# Autodesk Inventor assembly: Cycloidal Drive 1 - My Assembly
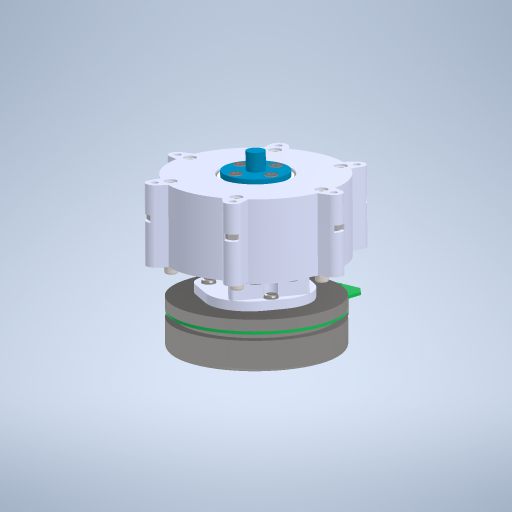
[picture p0: Inventor's stored thumbnail of the model, 512x512]
Saved by Autodesk Inventor 2023.2 (Build 272271000, 271)
## iProperties
Created: 2023-01-18
Part Number: Cycloidal Drive 1 - My Assembly
Document SubType Name: Assembly
Designer: Letícia
Author: Letícia
## Documents named in this file (31)
- C:\Users\User\Desktop\IC - Prof. Rafael\CADs\Redução Cicloidal\HowToMechatronics\Cycloidal Drive R25 - 3D\Cycloidal Drive - My Assembly.iam
- C:\Users\User\Desktop\IC - Prof. Rafael\CADs\Redução Cicloidal\HowToMechatronics\Cycloidal Drive R25 - 3D\Eccentric shaft v3.ipt
- C:\Users\User\Desktop\IC - Prof. Rafael\CADs\Redução Cicloidal\HowToMechatronics\Cycloidal Drive R25 - 3D\Ball Bearing-17x26x5mm.ipt
- C:\Users\User\Desktop\IC - Prof. Rafael\CADs\Redução Cicloidal\HowToMechatronics\Cycloidal Drive R25 - 3D\Ball Bearing-15x24x5mm 1.ipt
- C:\Users\User\Desktop\IC - Prof. Rafael\CADs\Redução Cicloidal\HowToMechatronics\Cycloidal Drive R25 - 3D\Distance ring 2.ipt
- C:\Users\User\Desktop\IC - Prof. Rafael\CADs\Redução Cicloidal\HowToMechatronics\Cycloidal Drive R25 - 3D\Cycloidal Disk v3 -.ipt
- C:\Users\User\Desktop\IC - Prof. Rafael\CADs\Redução Cicloidal\HowToMechatronics\Cycloidal Drive R25 - 3D\Output shaft p1 v3.ipt
- C:\Users\User\Desktop\IC - Prof. Rafael\CADs\Redução Cicloidal\HowToMechatronics\Cycloidal Drive R25 - 3D\Output shaft v3.ipt
- C:\Users\User\Desktop\IC - Prof. Rafael\CADs\Redução Cicloidal\HowToMechatronics\Cycloidal Drive R25 - 3D\Bushing 6x8mm.ipt
- C:\Users\User\Desktop\IC - Prof. Rafael\CADs\Redução Cicloidal\HowToMechatronics\Cycloidal Drive R25 - 3D\Pin 6x22mm r1.ipt
- C:\Users\User\Desktop\IC - Prof. Rafael\CADs\Redução Cicloidal\HowToMechatronics\Cycloidal Drive R25 - 3D\Input shaft 1 v3.ipt
- C:\Users\User\Desktop\IC - Prof. Rafael\CADs\Redução Cicloidal\HowToMechatronics\Cycloidal Drive R25 - 3D\Threaded insert M3 v3.ipt
- C:\Users\User\Desktop\IC - Prof. Rafael\CADs\Redução Cicloidal\HowToMechatronics\Cycloidal Drive R25 - 3D\porca prisioneiro.ipt
- C:\Users\User\Desktop\IC - Prof. Rafael\CADs\Redução Cicloidal\HowToMechatronics\Cycloidal Drive R25 - 3D\parafuso prisioneiro.ipt
- C:\Users\User\Desktop\IC - Prof. Rafael\CADs\Redução Cicloidal\HowToMechatronics\Cycloidal Drive R25 - 3D\EN ISO 4762 M3 x 25 - 18N_EN ISO 4762 M3 x 25 - 18N.ipt
- C:\Users\User\Desktop\IC - Prof. Rafael\CADs\Redução Cicloidal\HowToMechatronics\Cycloidal Drive R25 - 3D\Base housing.ipt
- C:\Users\User\Desktop\IC - Prof. Rafael\CADs\Redução Cicloidal\HowToMechatronics\Cycloidal Drive R25 - 3D\Pin 6x30mm r1.ipt
- C:\Users\User\Desktop\IC - Prof. Rafael\CADs\Redução Cicloidal\HowToMechatronics\Cycloidal Drive R25 - 3D\Ball Bearing-35x47x7mm 2.ipt
- C:\Users\User\Desktop\IC - Prof. Rafael\CADs\Redução Cicloidal\HowToMechatronics\Cycloidal Drive R25 - 3D\Housing lid.ipt
- C:\Users\User\Desktop\IC - Prof. Rafael\CADs\Redução Cicloidal\HowToMechatronics\Cycloidal Drive R25 - 3D\EN ISO 4762 M4 x 40 - 20N_EN ISO 4762 M4 x 40 - 20N.ipt
- C:\Users\User\Desktop\IC - Prof. Rafael\CADs\Redução Cicloidal\HowToMechatronics\Cycloidal Drive R25 - 3D\Distance ring for rollers bushings.ipt
- C:\Users\User\Desktop\IC - Prof. Rafael\CADs\Redução Cicloidal\HowToMechatronics\Cycloidal Drive R25 - 3D\DIN EN ISO 10511 - M4 - N_DIN EN ISO 10511 - M4 - N.ipt
- C:\Users\User\Desktop\IC - Prof. Rafael\CADs\Redução Cicloidal\HowToMechatronics\Cycloidal Drive R25 - 3D\MAXON motor mount v1.ipt
- C:\Users\User\Desktop\IC - Prof. Rafael\CADs\Redução Cicloidal\HowToMechatronics\Cycloidal Drive R25 - 3D\Threaded insert M4 - L5mm.ipt
- C:\Users\User\Desktop\IC - Prof. Rafael\Bancada\Motor Maxon323772_EC90fl_90W_A.ipt
- C:\Users\User\Documents\Inventor\Content Center Files\R2023\pt-BR\JIS B 1174\JIS B 1174 - M4 x 8.ipt
- C:\Users\User\Documents\Inventor\Content Center Files\R2023\pt-BR\ISO 4035(1)\ISO 4035 - M4DIN EN.ipt
- C:\Users\User\Desktop\IC - Prof. Rafael\CADs\Redução Cicloidal\HowToMechatronics\Cycloidal Drive R25 - 3D\eixo saida.ipt
- C:\Users\User\Documents\Inventor\Content Center Files\R2023\pt-BR\AS 1427(04)\AS 1427 - M4 x 8(5) I.ipt
- C:\Users\User\Documents\Inventor\Content Center Files\R2023\pt-BR\DIN 7991(2)\DIN 7991 - M4x8.ipt
- C:\Users\User\Desktop\IC - Prof. Rafael\CADs\Redução Cicloidal\HowToMechatronics\Cycloidal Drive R25 - 3D\Porca M4.ipt
## Components (157 placed, 30 different names)
1. Eccentric shaft v3:1 — Coincidente:1, Coincidente:2, Coincidente:3, Coincidente:5, Coincidente:7, Coincidente:8, Coincidente:9, Coincidente:11, Coincidente:13, Coincidente:32, Coincidente:33, Coincidente:34, Coincidente:35, Coincidente:36
2. Ball Bearing-17x26x5mm:1 — Coincidente:5, Coincidente:6, Coincidente:15, Alinhado:2
3. Ball Bearing-17x26x5mm:2 — Coincidente:7, Coincidente:8, Coincidente:14, Alinhado:1
4. Ball Bearing-15x24x5mm 1:1 — Coincidente:3, Coincidente:4, Coincidente:19, Coincidente:20
5. Distance ring 2:1 — Coincidente:1, Coincidente:2, Coincidente:4, Coincidente:6
6. Cycloidal Disk v3 -:1 — Coincidente:15, Alinhado:2, Coincidente:16
7. Cycloidal Disk v3 -:2 — Coincidente:14, Alinhado:1, Coincidente:16, Coincidente:21, Coincidente:22
8. Ball Bearing-15x24x5mm 1:2 — Coincidente:11, Coincidente:12, Coincidente:17, Coincidente:18
9. Distance ring 2:2 — Coincidente:9, Coincidente:12, Coincidente:13
10. Output shaft p1 v3:1 — Coincidente:17, Coincidente:18, Coincidente:21, Coincidente:44
11. Output shaft v3:1 — Coincidente:19, Coincidente:20, Coincidente:22, Coincidente:25, Alinhado:3, Coincidente:43, Coincidente:54, Coincidente:76, Inserir:10, Inserir:11, Inserir:12, Inserir:13, Coincidente:80
12. Input shaft 1 v3:1 — Coincidente:26, Coincidente:27, Coincidente:32, Coincidente:33, Coincidente:62, Coincidente:63, Coincidente:64, Coincidente:66, Coincidente:68
13. Base housing:1 — Coincidente:37, Coincidente:38, Coincidente:39, Coincidente:41, Coincidente:42, Coincidente:56, Coincidente:57, Coincidente:58, Coincidente:61, Coincidente:67, Coincidente:69, Coincidente:70, Coincidente:71, Coincidente:73, Coincidente:74, Coincidente:75, Alinhado:4, Alinhado:5, Alinhado:6, Alinhado:7, Coincidente:89, Coincidente:90
14. Ball Bearing-35x47x7mm 2:1 — Coincidente:41, Coincidente:42, Coincidente:43, Coincidente:44
15. Housing lid:1 — Coincidente:45, Coincidente:46, Coincidente:47, Coincidente:48, Coincidente:56, Coincidente:57, Coincidente:59
16. Ball Bearing-35x47x7mm 2:2 — Coincidente:47, Coincidente:48, Coincidente:76, Coincidente:81
17. Distance ring for rollers bushings:1 — Coincidente:54, Coincidente:55
18. MAXON motor mount v1:1 — Coincidente:67, Coincidente:68, Coincidente:69, Coincidente:70, Coincidente:77, Coincidente:78, Coincidente:79, Inserir:7, Inserir:8, Inserir:9, Coincidente:85, Coincidente:86, Coincidente:87, Coincidente:88
19. Threaded insert M4 - L5mm:1 — Coincidente:71, Alinhado:7
20. Threaded insert M4 - L5mm:2 — Coincidente:73, Alinhado:6
21. Threaded insert M4 - L5mm:3 — Coincidente:74, Alinhado:5
22. Threaded insert M4 - L5mm:4 — Coincidente:75, Alinhado:4
23. Motor Maxon323772_EC90fl_90W_A:1 — Coincidente:77, Coincidente:78, Coincidente:79
24. JIS B 1174 - Métrica M4 x 8:2 — Inserir:7
25. JIS B 1174 - Métrica M4 x 8:3 — Inserir:8
26. JIS B 1174 - Métrica M4 x 8:4 — Inserir:9
27. DIN EN 24035 M4:2 — Inserir:10
28. DIN EN 24035 M4:3 — Inserir:11, Coincidente:82
29. DIN EN 24035 M4:4 — Inserir:12
30. DIN EN 24035 M4:5 — Inserir:13, Coincidente:83
31. eixo saida:1 — Coincidente:80, Coincidente:81, Coincidente:82, Coincidente:84
32. DIN 7991 M4x8:1 — Coincidente:85
33. DIN 7991 M4x8:2 — Coincidente:86
34. DIN 7991 M4x8:3 — Coincidente:87
35. DIN 7991 M4x8:4 — Coincidente:88
36. Pin 6x22mm r1:1 — Coincidente:23, Coincidente:24, Coincidente:25, Alinhado:3
37. Pin 6x22mm r1:2
38. Pin 6x22mm r1:3
39. Pin 6x22mm r1:4
40. Pin 6x22mm r1:5
41. Pin 6x22mm r1:6
42. Threaded insert M3 v3:1 — Coincidente:26, Coincidente:27
43. Threaded insert M3 v3:2
44. Threaded insert M3 v3:3 — Coincidente:34
45. EN ISO 4762 M3 x 25 - 18N_EN ISO 4762 M3 x 25 - 18N:1 — Coincidente:35, Coincidente:36
46. EN ISO 4762 M3 x 25 - 18N_EN ISO 4762 M3 x 25 - 18N:2
47. EN ISO 4762 M3 x 25 - 18N_EN ISO 4762 M3 x 25 - 18N:3
48. Bushing 6x8mm:2 — Coincidente:37, Coincidente:38, Coincidente:40
49. Bushing 6x8mm:3
50. Bushing 6x8mm:4
51. Bushing 6x8mm:5
52. Bushing 6x8mm:6
53. Bushing 6x8mm:7
54. Bushing 6x8mm:8
55. Bushing 6x8mm:9
56. Bushing 6x8mm:10
57. Bushing 6x8mm:11 — Coincidente:55
58. Bushing 6x8mm:12
59. Bushing 6x8mm:13
60. Bushing 6x8mm:14
61. Bushing 6x8mm:15
62. Bushing 6x8mm:16
63. Bushing 6x8mm:17
64. Bushing 6x8mm:18
65. Bushing 6x8mm:19
66. Bushing 6x8mm:20
67. Bushing 6x8mm:21
68. Bushing 6x8mm:22
69. Bushing 6x8mm:23
70. Bushing 6x8mm:24
71. Bushing 6x8mm:25
72. Bushing 6x8mm:26
73. Bushing 6x8mm:27
74. Pin 6x30mm r1:1 — Coincidente:39, Coincidente:40
75. Pin 6x30mm r1:2
76. Pin 6x30mm r1:3
77. Pin 6x30mm r1:4
78. Pin 6x30mm r1:5
79. Pin 6x30mm r1:6
80. Pin 6x30mm r1:7
81. Pin 6x30mm r1:8
82. Pin 6x30mm r1:9
83. Pin 6x30mm r1:10
84. Pin 6x30mm r1:11
85. Pin 6x30mm r1:12
86. Pin 6x30mm r1:13
87. Pin 6x30mm r1:14
88. Pin 6x30mm r1:15
89. Pin 6x30mm r1:16
90. Pin 6x30mm r1:17
91. Pin 6x30mm r1:18
92. Pin 6x30mm r1:19
93. Pin 6x30mm r1:20
94. Pin 6x30mm r1:21
95. Pin 6x30mm r1:22
96. Pin 6x30mm r1:23
97. Pin 6x30mm r1:24
98. Pin 6x30mm r1:25
99. Pin 6x30mm r1:26
100. Bushing 6x8mm:28 — Coincidente:45, Coincidente:46
101. Bushing 6x8mm:29
102. Bushing 6x8mm:30
103. Bushing 6x8mm:31
104. Bushing 6x8mm:32
105. Bushing 6x8mm:33
106. Bushing 6x8mm:34
107. Bushing 6x8mm:35
108. Bushing 6x8mm:36
109. Bushing 6x8mm:37
110. Bushing 6x8mm:38
111. Bushing 6x8mm:39
112. Bushing 6x8mm:40
113. Bushing 6x8mm:41
114. Bushing 6x8mm:42
115. Bushing 6x8mm:43
116. Bushing 6x8mm:44
117. Bushing 6x8mm:45
118. Bushing 6x8mm:46
119. Bushing 6x8mm:47
120. Bushing 6x8mm:48
121. Bushing 6x8mm:49
122. Bushing 6x8mm:50
123. Bushing 6x8mm:51
124. Bushing 6x8mm:52
125. Bushing 6x8mm:53
126. DIN EN ISO 10511 - M4 - N_DIN EN ISO 10511 - M4 - N:1 — Coincidente:60, Coincidente:61
127. EN ISO 4762 M4 x 40 - 20N_EN ISO 4762 M4 x 40 - 20N:1 — Coincidente:58, Coincidente:59, Coincidente:60
128. DIN EN ISO 10511 - M4 - N_DIN EN ISO 10511 - M4 - N:2
129. EN ISO 4762 M4 x 40 - 20N_EN ISO 4762 M4 x 40 - 20N:2
130. DIN EN ISO 10511 - M4 - N_DIN EN ISO 10511 - M4 - N:3
131. EN ISO 4762 M4 x 40 - 20N_EN ISO 4762 M4 x 40 - 20N:3
132. DIN EN ISO 10511 - M4 - N_DIN EN ISO 10511 - M4 - N:4
133. EN ISO 4762 M4 x 40 - 20N_EN ISO 4762 M4 x 40 - 20N:4
134. DIN EN ISO 10511 - M4 - N_DIN EN ISO 10511 - M4 - N:5
135. EN ISO 4762 M4 x 40 - 20N_EN ISO 4762 M4 x 40 - 20N:5
136. DIN EN ISO 10511 - M4 - N_DIN EN ISO 10511 - M4 - N:6
137. EN ISO 4762 M4 x 40 - 20N_EN ISO 4762 M4 x 40 - 20N:6
138. porca prisioneiro:1 — Coincidente:62, Coincidente:63, Coincidente:64, Coincidente:65
139. parafuso prisioneiro:1 — Coincidente:65, Coincidente:66
140. porca prisioneiro:2
141. parafuso prisioneiro:2
142. AS 1427 H - Métrica M4 x 8:1 — Coincidente:83, Coincidente:84
143. AS 1427 H - Métrica M4 x 8:2
144. AS 1427 H - Métrica M4 x 8:3
145. AS 1427 H - Métrica M4 x 8:4
146. Bushing 6x8mm:1 — Coincidente:23, Coincidente:24
147. Bushing 6x8mm:54
148. Bushing 6x8mm:55
149. Bushing 6x8mm:56
150. Bushing 6x8mm:57
151. Bushing 6x8mm:58
152. Porca M4:1 — Coincidente:89, Coincidente:90
153. Porca M4:2
154. Porca M4:3
155. Porca M4:4
156. Porca M4:5
157. Porca M4:6
## Component patterns: (6 elements, first: Pin 6x22mm r1:1), (3 elements, first: Threaded insert M3 v3:1), (3 elements, first: EN ISO 4762 M3 x 25 - 18N_EN ISO 4762 M3 x 25 - 18N:1), (26 elements, first: Bushing 6x8mm:2), (26 elements, first: Pin 6x30mm r1:1), (26 elements, first: Bushing 6x8mm:28), (6 elements, first: DIN EN ISO 10511 - M4 - N_DIN EN ISO 10511 - M4 - N:1 + EN ISO 4762 M4 x 40 - 20N_EN ISO 4762 M4 x 40 - 20N:1), (2 elements, first: porca prisioneiro:1 + parafuso prisioneiro:1), (4 elements, first: AS 1427 H - Métrica M4 x 8:1), (6 elements, first: Bushing 6x8mm:1), (6 elements, first: Porca M4:1)
## Relationships (93: Mate 79, Flush 7, Insert 7)
- Coincidente:1 [Mate]: Eccentric shaft v3:1 ↔ Distance ring 2:1
- Coincidente:2 [Mate]: Eccentric shaft v3:1 ↔ Distance ring 2:1
- Coincidente:3 [Mate]: Eccentric shaft v3:1 ↔ Ball Bearing-15x24x5mm 1:1
- Coincidente:4 [Mate]: Ball Bearing-15x24x5mm 1:1 ↔ Distance ring 2:1
- Coincidente:5 [Mate]: Eccentric shaft v3:1 ↔ Ball Bearing-17x26x5mm:1
- Coincidente:6 [Mate]: Ball Bearing-17x26x5mm:1 ↔ Distance ring 2:1
- Coincidente:7 [Mate]: Eccentric shaft v3:1 ↔ Ball Bearing-17x26x5mm:2
- Coincidente:8 [Mate]: Eccentric shaft v3:1 ↔ Ball Bearing-17x26x5mm:2
- Coincidente:9 [Mate]: Eccentric shaft v3:1 ↔ Distance ring 2:2
- Coincidente:11 [Mate]: Eccentric shaft v3:1 ↔ Ball Bearing-15x24x5mm 1:2
- Coincidente:12 [Mate]: Ball Bearing-15x24x5mm 1:2 ↔ Distance ring 2:2
- Coincidente:13 [Mate]: Eccentric shaft v3:1 ↔ Distance ring 2:2
- Coincidente:14 [Mate]: Ball Bearing-17x26x5mm:2 ↔ Cycloidal Disk v3 -:2
- Alinhado:1 [Flush]: Ball Bearing-17x26x5mm:2 ↔ Cycloidal Disk v3 -:2
- Coincidente:15 [Mate]: Ball Bearing-17x26x5mm:1 ↔ Cycloidal Disk v3 -:1
- Alinhado:2 [Flush]: Ball Bearing-17x26x5mm:1 ↔ Cycloidal Disk v3 -:1
- Coincidente:16 [Mate]: Cycloidal Disk v3 -:1 ↔ Cycloidal Disk v3 -:2
- Coincidente:17 [Mate]: Ball Bearing-15x24x5mm 1:2 ↔ Output shaft p1 v3:1
- Coincidente:18 [Mate]: Ball Bearing-15x24x5mm 1:2 ↔ Output shaft p1 v3:1
- Coincidente:19 [Mate]: Ball Bearing-15x24x5mm 1:1 ↔ Output shaft v3:1
- Coincidente:20 [Mate]: Ball Bearing-15x24x5mm 1:1 ↔ Output shaft v3:1
- Coincidente:21 [Mate]: Cycloidal Disk v3 -:2 ↔ Output shaft p1 v3:1
- Coincidente:22 [Mate]: Cycloidal Disk v3 -:2 ↔ Output shaft v3:1
- Coincidente:23 [Mate]: Pin 6x22mm r1:1 ↔ Bushing 6x8mm:1
- Coincidente:24 [Mate] (6 mm): Pin 6x22mm r1:1 ↔ Bushing 6x8mm:1
- Coincidente:25 [Mate]: Output shaft v3:1 ↔ Pin 6x22mm r1:1
- Alinhado:3 [Flush] (0.9 mm): Output shaft v3:1 ↔ Pin 6x22mm r1:1
- Coincidente:26 [Mate]: Input shaft 1 v3:1 ↔ Threaded insert M3 v3:1
- Coincidente:27 [Mate] (0.5 mm): Input shaft 1 v3:1 ↔ Threaded insert M3 v3:1
- Coincidente:32 [Mate]: Eccentric shaft v3:1 ↔ Input shaft 1 v3:1
- Coincidente:33 [Mate]: Eccentric shaft v3:1 ↔ Input shaft 1 v3:1
- Coincidente:34 [Mate]: Eccentric shaft v3:1 ↔ Threaded insert M3 v3:3
- Coincidente:35 [Mate]: Eccentric shaft v3:1 ↔ EN ISO 4762 M3 x 25 - 18N_EN ISO 4762 M3 x 25 - 18N:1
- Coincidente:36 [Mate]: Eccentric shaft v3:1 ↔ EN ISO 4762 M3 x 25 - 18N_EN ISO 4762 M3 x 25 - 18N:1
- Coincidente:37 [Mate]: Base housing:1 ↔ Bushing 6x8mm:2
- Coincidente:38 [Mate]: Base housing:1 ↔ Bushing 6x8mm:2
- Coincidente:39 [Mate]: Base housing:1 ↔ Pin 6x30mm r1:1
- Coincidente:40 [Mate]: Bushing 6x8mm:2 ↔ Pin 6x30mm r1:1
- Coincidente:41 [Mate]: Base housing:1 ↔ Ball Bearing-35x47x7mm 2:1
- Coincidente:42 [Mate]: Base housing:1 ↔ Ball Bearing-35x47x7mm 2:1
- Coincidente:43 [Mate]: Output shaft v3:1 ↔ Ball Bearing-35x47x7mm 2:1
- Coincidente:44 [Mate]: Output shaft p1 v3:1 ↔ Ball Bearing-35x47x7mm 2:1
- Coincidente:45 [Mate]: Housing lid:1 ↔ Bushing 6x8mm:28
- Coincidente:46 [Mate]: Housing lid:1 ↔ Bushing 6x8mm:28
- Coincidente:47 [Mate]: Housing lid:1 ↔ Ball Bearing-35x47x7mm 2:2
- Coincidente:48 [Mate]: Housing lid:1 ↔ Ball Bearing-35x47x7mm 2:2
- Coincidente:54 [Mate]: Output shaft v3:1 ↔ Distance ring for rollers bushings:1
- Coincidente:55 [Mate]: Distance ring for rollers bushings:1 ↔ Bushing 6x8mm:11
- Coincidente:56 [Mate]: Base housing:1 ↔ Housing lid:1
- Coincidente:57 [Mate]: Base housing:1 ↔ Housing lid:1
- Coincidente:58 [Mate]: Base housing:1 ↔ EN ISO 4762 M4 x 40 - 20N_EN ISO 4762 M4 x 40 - 20N:1
- Coincidente:59 [Mate]: Housing lid:1 ↔ EN ISO 4762 M4 x 40 - 20N_EN ISO 4762 M4 x 40 - 20N:1
- Coincidente:60 [Mate]: DIN EN ISO 10511 - M4 - N_DIN EN ISO 10511 - M4 - N:1 ↔ EN ISO 4762 M4 x 40 - 20N_EN ISO 4762 M4 x 40 - 20N:1
- Coincidente:61 [Mate]: Base housing:1 ↔ DIN EN ISO 10511 - M4 - N_DIN EN ISO 10511 - M4 - N:1
- Coincidente:62 [Mate]: Input shaft 1 v3:1 ↔ porca prisioneiro:1
- Coincidente:63 [Mate]: Input shaft 1 v3:1 ↔ porca prisioneiro:1
- Coincidente:64 [Mate]: Input shaft 1 v3:1 ↔ porca prisioneiro:1
- Coincidente:65 [Mate]: porca prisioneiro:1 ↔ parafuso prisioneiro:1
- Coincidente:66 [Mate] (4 mm): Input shaft 1 v3:1 ↔ parafuso prisioneiro:1
- Coincidente:67 [Mate]: Base housing:1 ↔ MAXON motor mount v1:1
- Coincidente:68 [Mate]: Input shaft 1 v3:1 ↔ MAXON motor mount v1:1
- Coincidente:69 [Mate]: Base housing:1 ↔ MAXON motor mount v1:1
- Coincidente:70 [Mate]: Base housing:1 ↔ MAXON motor mount v1:1
- Coincidente:71 [Mate]: Base housing:1 ↔ Threaded insert M4 - L5mm:1
- Coincidente:73 [Mate]: Base housing:1 ↔ Threaded insert M4 - L5mm:2
- Coincidente:74 [Mate]: Base housing:1 ↔ Threaded insert M4 - L5mm:3
- Coincidente:75 [Mate]: Base housing:1 ↔ Threaded insert M4 - L5mm:4
- Alinhado:4 [Flush]: Base housing:1 ↔ Threaded insert M4 - L5mm:4
- Alinhado:5 [Flush]: Base housing:1 ↔ Threaded insert M4 - L5mm:3
- Alinhado:6 [Flush]: Base housing:1 ↔ Threaded insert M4 - L5mm:2
- Alinhado:7 [Flush]: Base housing:1 ↔ Threaded insert M4 - L5mm:1
- Coincidente:76 [Mate]: Output shaft v3:1 ↔ Ball Bearing-35x47x7mm 2:2
- Coincidente:77 [Mate]: MAXON motor mount v1:1 ↔ Motor Maxon323772_EC90fl_90W_A:1
- Coincidente:78 [Mate]: MAXON motor mount v1:1 ↔ Motor Maxon323772_EC90fl_90W_A:1
- Coincidente:79 [Mate]: MAXON motor mount v1:1 ↔ Motor Maxon323772_EC90fl_90W_A:1
- Inserir:7: MAXON motor mount v1:1 ↔ JIS B 1174 - Métrica M4 x 8:2
- Inserir:8: MAXON motor mount v1:1 ↔ JIS B 1174 - Métrica M4 x 8:3
- Inserir:9: MAXON motor mount v1:1 ↔ JIS B 1174 - Métrica M4 x 8:4
- Inserir:10: Output shaft v3:1 ↔ DIN EN 24035 M4:2
- Inserir:11: Output shaft v3:1 ↔ DIN EN 24035 M4:3
- Inserir:12: Output shaft v3:1 ↔ DIN EN 24035 M4:4
- Inserir:13: Output shaft v3:1 ↔ DIN EN 24035 M4:5
- Coincidente:80 [Mate]: Output shaft v3:1 ↔ eixo saida:1
- Coincidente:81 [Mate]: Ball Bearing-35x47x7mm 2:2 ↔ eixo saida:1
- Coincidente:82 [Mate]: DIN EN 24035 M4:3 ↔ eixo saida:1
- Coincidente:83 [Mate]: DIN EN 24035 M4:5 ↔ AS 1427 H - Métrica M4 x 8:1
- Coincidente:84 [Mate]: eixo saida:1 ↔ AS 1427 H - Métrica M4 x 8:1
- Coincidente:85 [Mate]: MAXON motor mount v1:1 ↔ DIN 7991 M4x8:1
- Coincidente:86 [Mate]: MAXON motor mount v1:1 ↔ DIN 7991 M4x8:2
- Coincidente:87 [Mate]: MAXON motor mount v1:1 ↔ DIN 7991 M4x8:3
- Coincidente:88 [Mate]: MAXON motor mount v1:1 ↔ DIN 7991 M4x8:4
- Coincidente:89 [Mate]: Base housing:1 ↔ Porca M4:1
- Coincidente:90 [Mate]: Base housing:1 ↔ Porca M4:1
